# Autodesk Inventor assembly: Hourglass
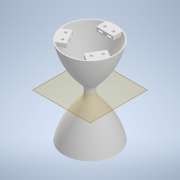
[picture p0: Inventor's stored thumbnail of the model, 180x180]
Saved by Autodesk Inventor 2020.2 (Build 242310000, 310)
## iProperties
Created: 2020-03-04
Part Number: Hourglass
Document SubType Name: Assembly
Designer: linus
Author: linus
## Documents named in this file (3)
- C:\Users\linus\Documents\Projects\Timglas\Hourglass.iam
- C:\Users\linus\Documents\Projects\Timglas\Timglas_main.ipt
- C:\Users\linus\Documents\Projects\Timglas\Top_and_Bottom.ipt
## Components (2 placed, 2 different names)
1. Timglas_main:1 — Flush:1
2. Top_and_Bottom:1 — Flush:1
## Relationships (1: Flush 1)
- Flush:1: Timglas_main:1 ↔ Top_and_Bottom:1
